# Autodesk Inventor assembly: ASY SLM 1690 Filter legs D1000
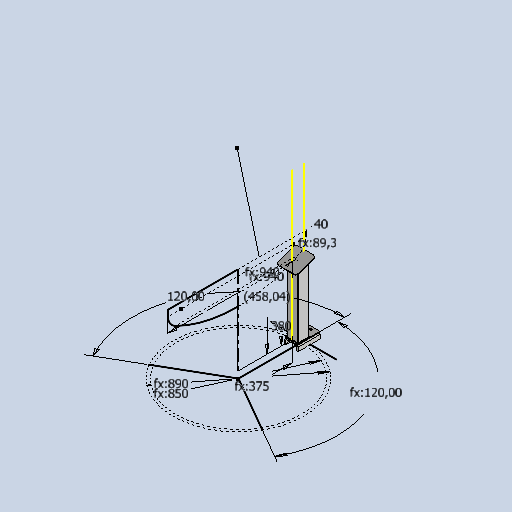
[picture p0: Inventor's stored thumbnail of the model, 512x512]
Saved by Autodesk Inventor 2025.3 (Build 293356030, 356C)
## iProperties
Created: 2025-02-20
Part Number: ASY SLM 1690 Filter legs D1000
Document SubType Name: Assembly
Designer: user
Mass: 20950.1 g
Surface Area: 14148.6 cm^2
Volume: 2651.55 cm^3
Density: 7.9011 g/cm^3
Author: user
## Documents named in this file (7)
- C:\Users\admin\Documents\Inventor\SLM-Salemal\ASY PNS 1690 Filter legs D1000.iam
- C:\Users\admin\Documents\Inventor\SLM-Salemal\PNS 1692 Leg tube.ipt
- C:\Users\admin\Documents\Inventor\SLM-Salemal\PNS 1693 leg sketch.ipt
- C:\Users\admin\Documents\Inventor\SLM-Salemal\PNS 1694 leg plate for filter.ipt
- C:\Users\admin\Documents\Inventor\SLM-Salemal\PNS 1695 leg floor plate.ipt
- C:\Users\admin\Documents\Inventor\SLM-Salemal\PNS 1785 leg floor channel.ipt
- C:\Users\admin\Documents\Inventor\SLM-Salemal\PNS 1696 leg floor pattern.ipt
## Components (6 placed, 6 different names)
1. PNS 1692 Leg tube.ipt:2 — Mate:4, Mate:5, Flush:1, Mate:6, Mate:7
2. PNS 1693 leg sketch.ipt:1 — Mate:6
3. PNS 1694 leg plate for filter.ipt:1 — Mate:7
4. PNS 1695 leg floor plate.ipt:1 — Rigid:10, Mate:5, Flush:1
5. PNS 1785 leg floor channel.ipt:1 — Rigid:10, Mate:1, Mate:2, Mate:8, Flush:2
6. PNS 1696 leg floor pattern.ipt:1 — Mate:8, Flush:2, Flush:3
## Relationships (11: Mate 7, Flush 3, WeldJoint 1)
- Rigid:10 [WeldJoint]: PNS 1695 leg floor plate.ipt:1 ↔ PNS 1785 leg floor channel.ipt:1
- Mate:1: PNS 1785 leg floor channel.ipt:1
- Mate:2: PNS 1785 leg floor channel.ipt:1
- Mate:4: PNS 1692 Leg tube.ipt:2
- Mate:5: PNS 1692 Leg tube.ipt:2 ↔ PNS 1695 leg floor plate.ipt:1
- Flush:1 (5 mm): PNS 1692 Leg tube.ipt:2 ↔ PNS 1695 leg floor plate.ipt:1
- Mate:6: PNS 1692 Leg tube.ipt:2 ↔ PNS 1693 leg sketch.ipt:1
- Mate:7: PNS 1692 Leg tube.ipt:2 ↔ PNS 1694 leg plate for filter.ipt:1
- Mate:8: PNS 1785 leg floor channel.ipt:1 ↔ PNS 1696 leg floor pattern.ipt:1
- Flush:2: PNS 1785 leg floor channel.ipt:1 ↔ PNS 1696 leg floor pattern.ipt:1
- Flush:3: PNS 1696 leg floor pattern.ipt:1
## Named parameters: Out_diam = 963 mm
